# Autodesk Inventor assembly: Motor_Section_Regular_Spacer
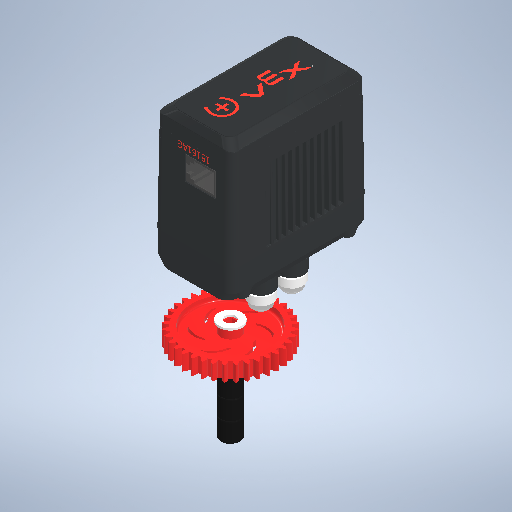
[picture p0: Inventor's stored thumbnail of the model, 512x512]
Saved by Autodesk Inventor 2025 (Build 290162000, 162)
## iProperties
Created: 2024-12-08
Part Number: Motor_Section_Regular_Spacer
Document SubType Name: Assembly
Designer: Aditya Koduri
Author: Aditya Koduri
## Documents named in this file (11)
- C:\Users\mzart\Downloads\Full_Cad_Model\Motor_Section_Regular_Spacer.iam
- C:\Users\mzart\Downloads\VEX-CAD-Inventor-main\VEX-CAD-Inventor-main\Motion\Spacers\Washer Teflon\TWasher .375 OD x .03125.ipt
- C:\Users\mzart\Downloads\VEX-CAD-Inventor-main\VEX-CAD-Inventor-main\Motion\Gears\LS 36T Gear.ipt
- C:\Users\mzart\Downloads\VEX-CAD-Inventor-main\VEX-CAD-Inventor-main\Electronics\V5 Motor.ipt
- C:\Users\mzart\Downloads\VEX-CAD-Inventor-main\VEX-CAD-Inventor-main\Motion\Spacers\Spacer Nylon .313 OD\NSpacer .313 OD x .125.ipt
- C:\Users\mzart\Downloads\VEX-CAD-Inventor-main\VEX-CAD-Inventor-main\Structure\Hardware\Screw Steel - Hex\SScrew Hex Smooth .500.ipt
- C:\Users\mzart\Downloads\VEX-CAD-Inventor-main\VEX-CAD-Inventor-main\Motion\Spacers\Spacer Plastic\PSpacer 8.0.ipt
- C:\Users\mzart\Downloads\VEX-CAD-Inventor-main\VEX-CAD-Inventor-main\Motion\Spacers\Washer Teflon.ipt
- C:\Users\mzart\Downloads\VEX-CAD-Inventor-main\VEX-CAD-Inventor-main\Motion\Spacers\Spacer Nylon .313 OD.ipt
- C:\Users\mzart\Downloads\VEX-CAD-Inventor-main\VEX-CAD-Inventor-main\Motion\Spacers\Spacer Plastic.ipt
- C:\Users\mzart\Downloads\VEX-CAD-Inventor-main\VEX-CAD-Inventor-main\Structure\Hardware\Screw Steel - Hex.ipt
## Components (11 placed, 6 different names)
1. TWasher .375 OD x .03125:1
2. LS 36T Gear:1 — Insert:11
3. V5 Motor:1
4. NSpacer .313 OD x .125:1
5. NSpacer .313 OD x .125:2
6. SScrew Hex Smooth .500:1
7. SScrew Hex Smooth .500:2
8. PSpacer 8.0:1 — Insert:8, Insert:9
9. PSpacer 8.0:2 — Insert:8, Insert:10
10. PSpacer 8.0:3 — Insert:9, Insert:11
11. PSpacer 8.0:4 — Insert:10
## Relationships (7: Insert 7)
- [Insert]: TWasher .375 OD x .03125:1 ↔ LS 36T Gear:1
- [Insert]: V5 Motor:1 ↔ NSpacer .313 OD x .125:1
- [Insert]: V5 Motor:1 ↔ NSpacer .313 OD x .125:2
- Insert:8: PSpacer 8.0:1 ↔ PSpacer 8.0:2
- Insert:9: PSpacer 8.0:1 ↔ PSpacer 8.0:3
- Insert:10: PSpacer 8.0:2 ↔ PSpacer 8.0:4
- Insert:11: LS 36T Gear:1 ↔ PSpacer 8.0:3
